# Autodesk Inventor assembly: 34 tooth gear for 8 mm shaft
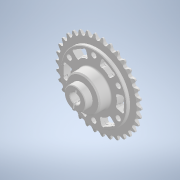
[picture p0: Inventor's stored thumbnail of the model, 180x180]
Saved by Autodesk Inventor 2020 (Build 240168000, 168)
## iProperties
Created: 2020-02-02
Part Number: 34 tooth gear for 8 mm shaft
Document SubType Name: Assembly
Designer: JimAndVal
Author: JimAndVal
## Documents named in this file (4)
- D:\Users\JimAndVal\Documents\JIM\IronRiders\2020 Robot-1\Manipulators\Hooded Shooter (Protected Zone)\34 tooth gear for 8 mm shaft.iam
- D:\Users\JimAndVal\Documents\JIM\IronRiders\2020 Robot-1\Manipulators\Hooded Shooter (Protected Zone)\Clamping_Shaft_Collar_-_8mm_Round_ID_217-2744.ipt
- D:\Users\JimAndVal\Documents\JIM\IronRiders\2020 Robot-1\Manipulators\Hooded Shooter (Protected Zone)\1_2_ID_1_8_Keyway_Aluminum_VersaHub_217-2590.ipt
- D:\Users\JimAndVal\Documents\JIM\IronRiders\2020 Robot-1\Manipulators\Hooded Shooter (Protected Zone)\_34t_Aluminum_Plate_Sprocket_25_Chain_1-1_8_Bearing_Bore_217-2664.ipt
## Components (4 placed, 3 different names)
1. Clamping_Shaft_Collar_-_8mm_Round_ID_217-2744:1 — Mate:5, Mate:6
2. Clamping_Shaft_Collar_-_8mm_Round_ID_217-2744:2 — Mate:3, Mate:4
3. 1_2_ID_1_8_Keyway_Aluminum_VersaHub_217-2590:1 — Mate:1, Mate:2, Mate:3, Mate:4, Mate:5, Mate:6
4. _34t_Aluminum_Plate_Sprocket_25_Chain_1-1_8_Bearing_Bore_217-2664:1 — Mate:1, Mate:2
## Relationships (6: Mate 6)
- Mate:1: 1_2_ID_1_8_Keyway_Aluminum_VersaHub_217-2590:1 ↔ _34t_Aluminum_Plate_Sprocket_25_Chain_1-1_8_Bearing_Bore_217-2664:1
- Mate:2: 1_2_ID_1_8_Keyway_Aluminum_VersaHub_217-2590:1 ↔ _34t_Aluminum_Plate_Sprocket_25_Chain_1-1_8_Bearing_Bore_217-2664:1
- Mate:3: Clamping_Shaft_Collar_-_8mm_Round_ID_217-2744:2 ↔ 1_2_ID_1_8_Keyway_Aluminum_VersaHub_217-2590:1
- Mate:4: Clamping_Shaft_Collar_-_8mm_Round_ID_217-2744:2 ↔ 1_2_ID_1_8_Keyway_Aluminum_VersaHub_217-2590:1
- Mate:5: Clamping_Shaft_Collar_-_8mm_Round_ID_217-2744:1 ↔ 1_2_ID_1_8_Keyway_Aluminum_VersaHub_217-2590:1
- Mate:6: Clamping_Shaft_Collar_-_8mm_Round_ID_217-2744:1 ↔ 1_2_ID_1_8_Keyway_Aluminum_VersaHub_217-2590:1
